# Autodesk Inventor assembly: Scrambler II
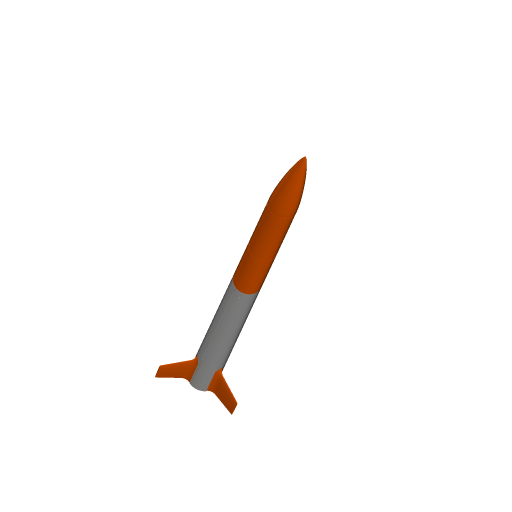
[picture p0: Inventor's stored thumbnail of the model, 512x512]
Saved by Autodesk Inventor 2024 (Build 280153000, 153)
## iProperties
Created: 2023-12-30
Part Number: Scrambler II
Document SubType Name: Assembly
Designer: Jamie
Mass: 631.455 g
Surface Area: 5625.65 cm^2
Volume: 391.502 cm^3
Density: 1.6129 g/cm^3
Author: Jamie
## Documents named in this file (8)
- C:\Users\Jamie\Documents\Uni\DARE\Scrambler-2-CAD\Autodesk\Scrambler II.iam
- C:\Users\Jamie\Documents\Uni\DARE\Scrambler-2-CAD\Autodesk\Structure.iam
- C:\Users\Jamie\Documents\Uni\DARE\Scrambler-2-CAD\Autodesk\Lower skin.ipt
- C:\Users\Jamie\Documents\Uni\DARE\Scrambler-2-CAD\Autodesk\Upper skin.ipt
- C:\Users\Jamie\Documents\Uni\DARE\Scrambler-2-CAD\Autodesk\SRM with Smoke Grain.iam
- C:\Users\Jamie\Documents\Uni\DARE\Scrambler-2-CAD\Autodesk\Nose assembly.iam
- C:\Users\Jamie\Documents\Uni\DARE\Scrambler-2-CAD\Autodesk\Runcam.ipt
- C:\Users\Jamie\Documents\Uni\DARE\Scrambler-2-CAD\Autodesk\Engine retention.ipt
## Components (7 placed, 7 different names)
1. Structure:1 [sub-assembly] — Mate:1, Mate:2, Mate:3, Mate:4, Mate:7, Mate:8, Mate:17, Mate:18, Mate:19, Mate:20, Mate:21
2. Lower skin:1 — Mate:1, Mate:2
3. Upper skin:1 — Mate:3, Mate:4, Mate:9, Mate:10, Mate:11
4. SRM with Smoke Grain:1 [sub-assembly] — Mate:7, Mate:8, Mate:16
5. Nose assembly:1 [sub-assembly] — Mate:9, Mate:10, Mate:11
6. Runcam:1 — Mate:19, Mate:20, Mate:21
7. Engine retention:1 — Mate:16, Mate:17, Mate:18
## Relationships (15: Mate 15)
- Mate:1: Structure:1 ↔ Lower skin:1
- Mate:2: Structure:1 ↔ Lower skin:1
- Mate:3: Structure:1 ↔ Upper skin:1
- Mate:4: Structure:1 ↔ Upper skin:1
- Mate:7: Structure:1 ↔ SRM with Smoke Grain:1
- Mate:8: Structure:1 ↔ SRM with Smoke Grain:1
- Mate:9: Upper skin:1 ↔ Nose assembly:1
- Mate:10: Upper skin:1 ↔ Nose assembly:1
- Mate:11: Upper skin:1 ↔ Nose assembly:1
- Mate:16: SRM with Smoke Grain:1 ↔ Engine retention:1
- Mate:17: Structure:1 ↔ Engine retention:1
- Mate:18: Structure:1 ↔ Engine retention:1
- Mate:19: Structure:1 ↔ Runcam:1
- Mate:20: Structure:1 ↔ Runcam:1
- Mate:21: Structure:1 ↔ Runcam:1
